# Autodesk Inventor assembly: Penthouse Assembly
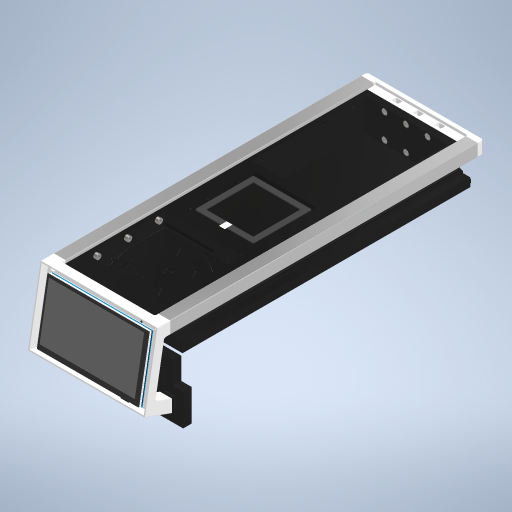
[picture p0: Inventor's stored thumbnail of the model, 512x512]
Saved by Autodesk Inventor 2024 (Build 280153000, 153)
## iProperties
Created: 2024-10-13
Part Number: Penthouse Assembly
Document SubType Name: Assembly
Designer: Ishaan
Author: Ishaan
## iProperties of the stored document PCBA Board.ipt
Created: 2024-10-16
Part Number: PCBA Board
Material: Generic
Document SubType Name: Modeling
Designer: Ishaan
Density: 1 g/cm^3
Appearance: Default
Author: Ishaan
Revision Number: ä»
## iProperties of the stored document 12X4_IC.ipt
Created: 2024-10-16
Part Number: 12X4_IC
Material: Generic
Document SubType Name: Modeling
Designer: Ishaan
Density: 1 g/cm^3
Appearance: Default
Author: Ishaan
Revision Number: ä»
## iProperties of the stored document ZIF Connector_50P.ipt
Created: 2024-10-16
Part Number: ZIF Connector_50P
Material: Generic
Document SubType Name: Modeling
Designer: Ishaan
Density: 1 g/cm^3
Appearance: Default
Author: Ishaan
Revision Number: ä»
## iProperties of the stored document Ras Pi 3B+.ipt
Created: 2021-02-26
Part Number: Ras Pi 3B+
Material: Generic
Description: STEP AP214
Document SubType Name: Modeling
Designer: Ishaan
Density: 1 g/cm^3
Appearance: Default
Sending System: SolidWorks 2020
Preprocessor: SwSTEP 2.0
Title: Ras Pi 3B+.STEP
Revision Number: ANY
## iProperties of the stored document 拨动开关.ipt
Created: 2024-10-16
Part Number: 拨动开关
Material: Generic
Document SubType Name: Modeling
Designer: Ishaan
Density: 1 g/cm^3
Appearance: Default
Author: Ishaan
Revision Number: ä»
## iProperties of the stored document ER-TFTV070A3-1.iam
Company: Î¢ÈíÖÐ¹ú
Created: 2024-07-16
Part Number: ER-TFTV070A3-1
Description: STEP AP214
Document SubType Name: Assembly
Designer: Ishaan
Sending System: SolidWorks 2023
Preprocessor: SwSTEP 2.0
Title: ER-TFTV070A3-1.STEP
Author: Î¢ÈíÓÃ»§
Revision Number: ä»
## iProperties of the stored document ER-TFT070A3-1_TFT 屏.ipt
Created: 2024-10-16
Part Number: ER-TFT070A3-1_TFT 屏
Material: Generic
Document SubType Name: Modeling
Designer: Ishaan
Density: 1 g/cm^3
Appearance: Default
Author: Ishaan
Revision Number: ä»
## iProperties of the stored document 15P连接器+IC.ipt
Created: 2024-10-16
Part Number: 15P连接器+IC
Material: Generic
Document SubType Name: Modeling
Designer: Ishaan
Density: 1 g/cm^3
Appearance: Default
Author: Ishaan
Revision Number: ä»
## iProperties of the stored document ZIF Connector_6P.ipt
Created: 2024-10-16
Part Number: ZIF Connector_6P
Material: Generic
Document SubType Name: Modeling
Designer: Ishaan
Density: 1 g/cm^3
Appearance: Default
Author: Ishaan
Revision Number: ä»
## Documents named in this file (23)
- E:\Projects\Axiom--IDEX-3D-Printer\CAD\09 - Penthouse\Penthouse Assembly.iam
- E:\Projects\Axiom--IDEX-3D-Printer\CAD\00 - COTS Components\2020 Penthouse Extrusions\HFST5-2020-500.ipt
- E:\Projects\Axiom--IDEX-3D-Printer\CAD\00 - COTS Components\HEPA Filter.ipt
- E:\Projects\Axiom--IDEX-3D-Printer\CAD\00 - COTS Components\Hardware\SHCSM5x12.ipt
- E:\Projects\Axiom--IDEX-3D-Printer\CAD\00 - COTS Components\Hardware\M5 T SLOT NUT.ipt
- E:\Projects\Axiom--IDEX-3D-Printer\CAD\00 - COTS Components\Hardware\SHCSM4x40.ipt
- E:\Projects\Axiom--IDEX-3D-Printer\CAD\00 - COTS Components\Hardware\M4 Shim.ipt
- E:\Projects\Axiom--IDEX-3D-Printer\CAD\00 - COTS Components\Hardware\M4 LOCKNUT.ipt
- **E:\Projects\Axiom--IDEX-3D-Printer\CAD\09 - Penthouse\Penthouse Assembly.iam*LocalDocs*xAaaaazcaAaaaaaaaAaaaajxoCa*ER-TFTV070A3-1.iam
- **E:\Projects\Axiom--IDEX-3D-Printer\CAD\09 - Penthouse\Penthouse Assembly.iam*LocalDocs*xAaaaaoaaAaaaaaaaAaaaa3rrTd*Ras Pi 3B+.ipt
- E:\Projects\Axiom--IDEX-3D-Printer\CAD\10 - Display Assembly\Display Cover.ipt
- E:\Projects\Axiom--IDEX-3D-Printer\CAD\09 - Penthouse\R2 Penthouse.ipt
- E:\Projects\Axiom--IDEX-3D-Printer\CAD\00 - COTS Components\12032 Fan\BFB1212\BFB1212L-F00\BFB1212L-F00.ipt
- E:\Projects\Axiom--IDEX-3D-Printer\CAD\00 - COTS Components\Hardware\SHCSM5x16.ipt
- **E:\Projects\Axiom--IDEX-3D-Printer\CAD\09 - Penthouse\Penthouse Assembly.iam*LocalDocs*xAaaaasdaAaaaaaaaAaaaamvoDd*PCBA Board.ipt
- **E:\Projects\Axiom--IDEX-3D-Printer\CAD\09 - Penthouse\Penthouse Assembly.iam*LocalDocs*xAaaaandaAaaaaaaaAaaaa5kzDb*12X4_IC.ipt
- **E:\Projects\Axiom--IDEX-3D-Printer\CAD\09 - Penthouse\Penthouse Assembly.iam*LocalDocs*xAaaaaabaAaaaaaaaAaaaq2zxRg*ZIF Connector_50P.ipt
- **E:\Projects\Axiom--IDEX-3D-Printer\CAD\09 - Penthouse\Penthouse Assembly.iam*LocalDocs*xAaaaqddaAaaaaaaaAaaaqja32h*拨动开关.ipt
- **E:\Projects\Axiom--IDEX-3D-Printer\CAD\09 - Penthouse\Penthouse Assembly.iam*LocalDocs*xAaaaqqdaAaaaaaaaAaaaa3lrGd*ER-TFT070A3-1_TFT 屏.ipt
- **E:\Projects\Axiom--IDEX-3D-Printer\CAD\09 - Penthouse\Penthouse Assembly.iam*LocalDocs*xAaaaqscaAaaaaaaaAaaaark0Of*ZIF Connector_6P.ipt
- **E:\Projects\Axiom--IDEX-3D-Printer\CAD\09 - Penthouse\Penthouse Assembly.iam*LocalDocs*xAaaaqgcaAaaaaaaaAaaaq22xBe*15P连接器+IC.ipt
- E:\Projects\Axiom--IDEX-3D-Printer\CAD\00 - COTS Components\Display Assem\ER-TFTV070A3-1.STEP
- E:\Projects\Axiom--IDEX-3D-Printer\CAD\00 - COTS Components\Pi 3B\Ras Pi 3B+.STEP
## Components (52 placed, 13 different names)
1. R2 Penthouse:1 — Insert:6, Insert:7, Insert:8, Insert:9, Insert:10, Insert:14, Insert:15, Insert:49, Insert:50, Insert:51, Insert:52, Insert:53, Insert:54, Insert:55, Insert:56, Insert:57
2. HFST5-2020-500:1 — Insert:47, Insert:52
3. HFST5-2020-500:2 — Insert:48
4. BFB1212L-F00:1 — Insert:39, Insert:40, Insert:41, Insert:49, Insert:50, Insert:51
5. HEPA Filter:1
6. ER-TFTV070A3-1:1 [sub-assembly] — Insert:45, Insert:46
7. Ras Pi 3B+:1 — Insert:45, Insert:46
8. Display Cover:1 — Insert:47, Insert:48
9. SHCSM5x12:16 — Insert:56
10. SHCSM5x12:17 — Insert:57
11. SHCSM5x16:1 — Insert:53
12. SHCSM5x16:2 — Insert:54
13. SHCSM5x16:3 — Insert:55
14. SHCSM4x40:1
15. SHCSM4x40:2
16. SHCSM4x40:3
17. M4 Shim:1 — Insert:41, Insert:44
18. M4 Shim:2 — Insert:40, Insert:43
19. M4 Shim:3 — Insert:39, Insert:42
20. M4 LOCKNUT:1 — Insert:44
21. M4 LOCKNUT:2 — Insert:43
22. M4 LOCKNUT:3 — Insert:42
23. SHCSM5x12:1 — Insert:10
24. SHCSM5x12:2 — Insert:9
25. SHCSM5x12:3 — Insert:6
26. SHCSM5x12:4 — Insert:7
27. SHCSM5x12:5 — Insert:8
28. M5 T SLOT NUT:1
29. M5 T SLOT NUT:2
30. M5 T SLOT NUT:3
31. M5 T SLOT NUT:4 — Insert:14
32. M5 T SLOT NUT:5 — Insert:15
33. SHCSM5x12:6
34. SHCSM5x12:7
35. SHCSM5x12:8
36. SHCSM5x12:9
37. SHCSM5x12:10
38. SHCSM5x12:11
39. SHCSM5x12:12
40. SHCSM5x12:13
41. SHCSM5x12:14
42. SHCSM5x12:15
43. M5 T SLOT NUT:6
44. M5 T SLOT NUT:7
45. M5 T SLOT NUT:8
46. M5 T SLOT NUT:9
47. M5 T SLOT NUT:10
48. M5 T SLOT NUT:11
49. M5 T SLOT NUT:12
50. M5 T SLOT NUT:13
51. M5 T SLOT NUT:14
52. M5 T SLOT NUT:15
## Relationships (73: Insert 52, Angle 15, Mate 5, Flush 1)
- [Mate]: R2 Penthouse:1 ↔ HEPA Filter:1
- [Mate] (0.5 mm): R2 Penthouse:1 ↔ HEPA Filter:1
- [Mate] (0.5 mm): R2 Penthouse:1 ↔ HEPA Filter:1
- Insert:6: R2 Penthouse:1 ↔ SHCSM5x12:3
- Insert:7: R2 Penthouse:1 ↔ SHCSM5x12:4
- Insert:8: R2 Penthouse:1 ↔ SHCSM5x12:5
- Insert:9: R2 Penthouse:1 ↔ SHCSM5x12:2
- Insert:10: R2 Penthouse:1 ↔ SHCSM5x12:1
- [Insert] (2 mm): R2 Penthouse:1 ↔ M5 T SLOT NUT:1
- [Insert] (2 mm): R2 Penthouse:1 ↔ M5 T SLOT NUT:3
- [Insert] (2 mm): R2 Penthouse:1 ↔ M5 T SLOT NUT:2
- [Angle] (0 deg): R2 Penthouse:1 ↔ M5 T SLOT NUT:2
- [Angle] (0 deg): R2 Penthouse:1 ↔ M5 T SLOT NUT:3
- [Angle] (0 deg): R2 Penthouse:1 ↔ M5 T SLOT NUT:1
- Insert:14 (2 mm): R2 Penthouse:1 ↔ M5 T SLOT NUT:4
- Insert:15 (2 mm): R2 Penthouse:1 ↔ M5 T SLOT NUT:5
- [Angle] (0 deg): R2 Penthouse:1 ↔ M5 T SLOT NUT:4
- [Angle] (0 deg): R2 Penthouse:1 ↔ M5 T SLOT NUT:5
- [Insert]: R2 Penthouse:1 ↔ SHCSM5x12:6
- [Insert]: R2 Penthouse:1 ↔ SHCSM5x12:7
- [Insert]: R2 Penthouse:1 ↔ SHCSM5x12:8
- [Insert]: R2 Penthouse:1 ↔ SHCSM5x12:9
- [Insert]: R2 Penthouse:1 ↔ SHCSM5x12:10
- [Insert]: R2 Penthouse:1 ↔ SHCSM5x12:11
- [Insert]: R2 Penthouse:1 ↔ SHCSM5x12:12
- [Insert]: R2 Penthouse:1 ↔ SHCSM5x12:13
- [Insert]: R2 Penthouse:1 ↔ SHCSM5x12:14
- [Insert]: R2 Penthouse:1 ↔ SHCSM5x12:15
- [Insert] (2 mm): R2 Penthouse:1 ↔ M5 T SLOT NUT:6
- [Insert] (2 mm): R2 Penthouse:1 ↔ M5 T SLOT NUT:7
- [Insert] (2 mm): R2 Penthouse:1 ↔ M5 T SLOT NUT:8
- [Insert] (2 mm): R2 Penthouse:1 ↔ M5 T SLOT NUT:9
- [Insert] (2 mm): R2 Penthouse:1 ↔ M5 T SLOT NUT:10
- [Angle] (0 deg): R2 Penthouse:1 ↔ M5 T SLOT NUT:6
- [Angle] (0 deg): R2 Penthouse:1 ↔ M5 T SLOT NUT:7
- [Angle] (0 deg): R2 Penthouse:1 ↔ M5 T SLOT NUT:8
- [Angle] (0 deg): R2 Penthouse:1 ↔ M5 T SLOT NUT:9
- [Angle] (0 deg): R2 Penthouse:1 ↔ M5 T SLOT NUT:10
- [Insert] (2 mm): R2 Penthouse:1 ↔ M5 T SLOT NUT:11
- [Insert] (2 mm): R2 Penthouse:1 ↔ M5 T SLOT NUT:12
- [Insert] (2 mm): R2 Penthouse:1 ↔ M5 T SLOT NUT:13
- [Insert] (2 mm): R2 Penthouse:1 ↔ M5 T SLOT NUT:14
- [Insert]: R2 Penthouse:1 ↔ M5 T SLOT NUT:15
- [Angle] (0 deg): R2 Penthouse:1 ↔ M5 T SLOT NUT:15
- [Angle] (0 deg): R2 Penthouse:1 ↔ M5 T SLOT NUT:14
- [Angle] (0 deg): R2 Penthouse:1 ↔ M5 T SLOT NUT:13
- [Angle] (0 deg): R2 Penthouse:1 ↔ M5 T SLOT NUT:12
- [Angle] (0 deg): R2 Penthouse:1 ↔ M5 T SLOT NUT:11
- [Insert]: R2 Penthouse:1 ↔ SHCSM4x40:3
- [Insert]: R2 Penthouse:1 ↔ SHCSM4x40:2
- [Insert]: R2 Penthouse:1 ↔ SHCSM4x40:1
- Insert:39: BFB1212L-F00:1 ↔ M4 Shim:3
- Insert:40: BFB1212L-F00:1 ↔ M4 Shim:2
- Insert:41: BFB1212L-F00:1 ↔ M4 Shim:1
- Insert:42: M4 Shim:3 ↔ M4 LOCKNUT:3
- Insert:43: M4 Shim:2 ↔ M4 LOCKNUT:2
- Insert:44: M4 Shim:1 ↔ M4 LOCKNUT:1
- Insert:45: ER-TFTV070A3-1:1 ↔ Ras Pi 3B+:1
- Insert:46: ER-TFTV070A3-1:1 ↔ Ras Pi 3B+:1
- [Mate] (0.2 mm): R2 Penthouse:1 ↔ HFST5-2020-500:1
- [Mate] (0.2 mm): R2 Penthouse:1 ↔ HFST5-2020-500:2
- [Flush] (4.25 mm): R2 Penthouse:1 ↔ HFST5-2020-500:2
- Insert:47 (0.2 mm): HFST5-2020-500:1 ↔ Display Cover:1
- Insert:48 (0.2 mm): HFST5-2020-500:2 ↔ Display Cover:1
- Insert:49: R2 Penthouse:1 ↔ BFB1212L-F00:1
- Insert:50: R2 Penthouse:1 ↔ BFB1212L-F00:1
- Insert:51: R2 Penthouse:1 ↔ BFB1212L-F00:1
- Insert:52 (0.2 mm): R2 Penthouse:1 ↔ HFST5-2020-500:1
- Insert:53: R2 Penthouse:1 ↔ SHCSM5x16:1
- Insert:54: R2 Penthouse:1 ↔ SHCSM5x16:2
- Insert:55: R2 Penthouse:1 ↔ SHCSM5x16:3
- Insert:56: R2 Penthouse:1 ↔ SHCSM5x12:16
- Insert:57: R2 Penthouse:1 ↔ SHCSM5x12:17
